# Autodesk Inventor assembly: 知能ロボコン540gia
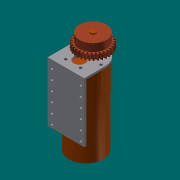
[picture p0: Inventor's stored thumbnail of the model, 180x180]
Saved by Autodesk Inventor 2013 (Build 170138000, 138)
## iProperties
Created: 2014-06-18
Part Number: 知能ロボコン540gia
Document SubType Name: Assembly
Designer: horumo136
Author: horumo136
## Documents named in this file (4)
- C:\Users\horumo136\Documents\知能ロボコン540gia.iam
- C:\Users\horumo136\Documents\知能ロボコンタミヤギヤードモータ540.ipt
- C:\Users\horumo136\Documents\平歯車.ipt
- C:\Users\horumo136\Documents\知能ロボコンタミヤギヤードモータ用マウント.ipt
## Components (3 placed, 3 different names)
1. 知能ロボコンタミヤギヤードモータ540:1 — メイト:4, メイト:5, メイト:6, メイト:7
2. 平歯車:1 — メイト:4
3. 知能ロボコンタミヤギヤードモータ用マウント:1 — メイト:5, メイト:6, メイト:7
## Relationships (4: Mate 4)
- メイト:4 [Mate]: 知能ロボコンタミヤギヤードモータ540:1 ↔ 平歯車:1
- メイト:5 [Mate]: 知能ロボコンタミヤギヤードモータ540:1 ↔ 知能ロボコンタミヤギヤードモータ用マウント:1
- メイト:6 [Mate]: 知能ロボコンタミヤギヤードモータ540:1 ↔ 知能ロボコンタミヤギヤードモータ用マウント:1
- メイト:7 [Mate]: 知能ロボコンタミヤギヤードモータ540:1 ↔ 知能ロボコンタミヤギヤードモータ用マウント:1
